# Autodesk Inventor assembly: Robot
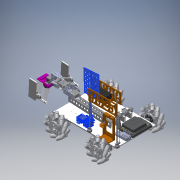
[picture p0: Inventor's stored thumbnail of the model, 180x180]
Saved by Autodesk Inventor 2017 (Build 210142000, 142)
## iProperties
Created: 2017-09-30
Part Number: Robot
Document SubType Name: Assembly
Designer: User
Author: User
## Documents named in this file (15)
- C:\Robotics\CAD\2017-18_CAD\Miscellaneous\Robot.iam
- C:\Robotics\CAD\2017-18_CAD\PlateFrame1.ipt
- C:\Robotics\CAD\2017-18_CAD\DirectDriveMotorSubAsembly.iam
- C:\Robotics\CAD\2017-18_CAD\batery.ipt
- C:\Robotics\CAD\2017-18_CAD\batteryholder.ipt
- C:\Robotics\CAD\2017-18_CAD\Miscellaneous\JewlArm.iam
- C:\Robotics\CAD\COTSParts\Tetrix\tetrix-motor-mounts-1.snapshot.1\Tetrex 2pc motor mount.ipt
- C:\Robotics\CAD\2017-18_CAD\MotorProtector.ipt
- C:\Robotics\CAD\2017-18_CAD\Numbers.ipt
- C:\Robotics\CAD\2017-18_CAD\FlapperSlapper.ipt
- C:\Robotics\CAD\2017-18_CAD\Phone_Cas.ipt
- C:\Robotics\CAD\2017-18_CAD\Miscellaneous\NewClawArm.iam
- C:\Robotics\CAD\2017-18_CAD\Miscellaneous\FlagHolder.ipt
- C:\Robotics\CAD\COTSParts\Rev\REV-31-1153RevHub.ipt
- C:\Robotics\CAD\COTSParts\Rev\REV-11-1144.ipt
## Components (19 placed, 14 different names)
1. PlateFrame1:1 — Mate:1, Mate:2, Mate:3, Mate:4, Mate:6, Mate:7, Mate:8, Mate:11, Mate:12, Mate:14, Mate:15, Mate:16, Mate:17, Mate:26, Mate:39, Mate:40, Flush:18, Flush:19, Flush:20, Flush:21, Mate:45, Flush:23, Flush:24, Flush:25, Mate:47, Flush:26, Flush:49, Mate:49, Mate:50, Flush:52, Flush:53, Mate:52, Mate:55, Mate:56, Mate:57, Flush:54, Flush:55, Mate:58, Flush:56
2. DirectDriveMotorSubAsembly:1 [sub-assembly] — Mate:1, Mate:2, Mate:3
3. DirectDriveMotorSubAsembly:3 [sub-assembly] — Mate:11, Mate:12, Mate:17
4. DirectDriveMotorSubAsembly:2 [sub-assembly] — Mate:14, Mate:15, Mate:16, Insert:1
5. DirectDriveMotorSubAsembly:4 [sub-assembly] — Mate:4, Mate:6, Mate:7, Mate:8
6. batery:1 — Mate:23, Mate:41, Mate:42
7. batteryholder:1 — Mate:23, Mate:26, Flush:18, Flush:19, Mate:41, Mate:42, Mate:46
8. JewlArm:1 [sub-assembly] — Mate:39, Flush:26, Flush:49
9. Tetrex 2pc motor mount:1 — Mate:40, Flush:20, Flush:21, Mate:53, Mate:54
10. MotorProtector:1 — Insert:1
11. Numbers:1 — Mate:45, Mate:46, Flush:23
12. Numbers:2 — Flush:24, Flush:25, Mate:47, Mate:48, Flush:50, Mate:51, Flush:51
13. FlapperSlapper:1 — Mate:50, Mate:51, Flush:51
14. FlapperSlapper:2 — Mate:48, Mate:49, Flush:50
15. Phone_Cas:1 — Flush:52, Flush:53, Mate:52
16. NewClawArm:2 [sub-assembly] — Mate:53, Mate:54, Mate:55
17. FlagHolder:1 — Mate:56
18. REV-31-1153RevHub:1 — Mate:57, Flush:54, Flush:55, Mate:59
19. REV-11-1144:1 — Mate:58, Flush:56, Mate:59
## Relationships (51: Mate 34, Flush 16, Insert 1)
- Mate:1: PlateFrame1:1 ↔ DirectDriveMotorSubAsembly:1
- Mate:2: PlateFrame1:1 ↔ DirectDriveMotorSubAsembly:1
- Mate:3: PlateFrame1:1 ↔ DirectDriveMotorSubAsembly:1
- Mate:4: PlateFrame1:1 ↔ DirectDriveMotorSubAsembly:4
- Mate:6: PlateFrame1:1 ↔ DirectDriveMotorSubAsembly:4
- Mate:7: PlateFrame1:1 ↔ DirectDriveMotorSubAsembly:4
- Mate:8: PlateFrame1:1 ↔ DirectDriveMotorSubAsembly:4
- Mate:11: PlateFrame1:1 ↔ DirectDriveMotorSubAsembly:3
- Mate:12: PlateFrame1:1 ↔ DirectDriveMotorSubAsembly:3
- Mate:14: PlateFrame1:1 ↔ DirectDriveMotorSubAsembly:2
- Mate:15: PlateFrame1:1 ↔ DirectDriveMotorSubAsembly:2
- Mate:16: PlateFrame1:1 ↔ DirectDriveMotorSubAsembly:2
- Mate:17: PlateFrame1:1 ↔ DirectDriveMotorSubAsembly:3
- Mate:23: batery:1 ↔ batteryholder:1
- Mate:26: PlateFrame1:1 ↔ batteryholder:1
- Mate:39 (12.7 mm): PlateFrame1:1 ↔ JewlArm:1
- Mate:40: PlateFrame1:1 ↔ Tetrex 2pc motor mount:1
- Flush:18 (1.5875 mm): PlateFrame1:1 ↔ batteryholder:1
- Flush:19 (19.05 mm): PlateFrame1:1 ↔ batteryholder:1
- Mate:41: batery:1 ↔ batteryholder:1
- Mate:42: batery:1 ↔ batteryholder:1
- Flush:20 (127 mm): PlateFrame1:1 ↔ Tetrex 2pc motor mount:1
- Flush:21 (-38.1 mm): PlateFrame1:1 ↔ Tetrex 2pc motor mount:1
- Insert:1: DirectDriveMotorSubAsembly:2 ↔ MotorProtector:1
- Mate:45: PlateFrame1:1 ↔ Numbers:1
- Mate:46: batteryholder:1 ↔ Numbers:1
- Flush:23: PlateFrame1:1 ↔ Numbers:1
- Flush:24: PlateFrame1:1 ↔ Numbers:2
- Flush:25: PlateFrame1:1 ↔ Numbers:2
- Mate:47 (190.5 mm): PlateFrame1:1 ↔ Numbers:2
- Flush:26 (152.4 mm): PlateFrame1:1 ↔ JewlArm:1
- Flush:49: PlateFrame1:1 ↔ JewlArm:1
- Mate:48: Numbers:2 ↔ FlapperSlapper:2
- Mate:49: PlateFrame1:1 ↔ FlapperSlapper:2
- Flush:50 (3.175 mm): Numbers:2 ↔ FlapperSlapper:2
- Mate:50: PlateFrame1:1 ↔ FlapperSlapper:1
- Mate:51: Numbers:2 ↔ FlapperSlapper:1
- Flush:51: Numbers:2 ↔ FlapperSlapper:1
- Flush:52: PlateFrame1:1 ↔ Phone_Cas:1
- Flush:53 (50.8 mm): PlateFrame1:1 ↔ Phone_Cas:1
- Mate:52: PlateFrame1:1 ↔ Phone_Cas:1
- Mate:53: Tetrex 2pc motor mount:1 ↔ NewClawArm:2
- Mate:54: Tetrex 2pc motor mount:1 ↔ NewClawArm:2
- Mate:55: PlateFrame1:1 ↔ NewClawArm:2
- Mate:56: PlateFrame1:1 ↔ FlagHolder:1
- Mate:57: PlateFrame1:1 ↔ REV-31-1153RevHub:1
- Flush:54: PlateFrame1:1 ↔ REV-31-1153RevHub:1
- Flush:55 (19.05 mm): PlateFrame1:1 ↔ REV-31-1153RevHub:1
- Mate:58: PlateFrame1:1 ↔ REV-11-1144:1
- Flush:56: PlateFrame1:1 ↔ REV-11-1144:1
- Mate:59 (6.35 mm): REV-31-1153RevHub:1 ↔ REV-11-1144:1
